# Autodesk Inventor assembly: 001_pakutta_all
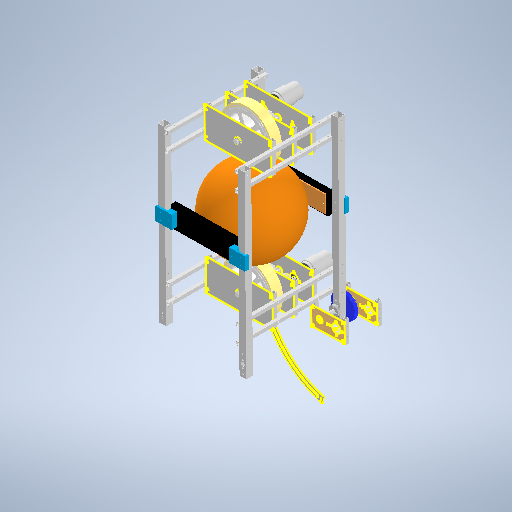
[picture p0: Inventor's stored thumbnail of the model, 512x512]
Saved by Autodesk Inventor 2025.1 (Build 291241000, 241)
## iProperties
Created: 2024-10-08
Part Number: 001_pakutta_all
Document SubType Name: Assembly
Designer: yuki0520
Author: yuki0520
## Documents named in this file (15)
- C:\Users\yuki0520\OneDrive\ドキュメント\Inventor\2025_nhk\tanaka\nageru\pakuriz\001_pakutta_all.iam
- C:\Users\yuki0520\OneDrive\ドキュメント\Inventor\2025_nhk\tanaka\nageru\pakuriz\001_pakutta_L.iam
- C:\Users\yuki0520\OneDrive\ドキュメント\Inventor\2025_nhk\tanaka\nageru\pakuriz\kaku_1010_530.ipt
- C:\Users\yuki0520\OneDrive\ドキュメント\Inventor\2025_nhk\tanaka\object\ball.ipt
- C:\Users\yuki0520\OneDrive\ドキュメント\Inventor\2025_nhk\tanaka\nageru\pakuriz\TH22_soroban_sn.ipt
- C:\Users\yuki0520\OneDrive\ドキュメント\Inventor\2025_nhk\tanaka\nageru\pakuriz\soroban_hold.ipt
- C:\Users\yuki0520\OneDrive\ドキュメント\Inventor\2025_nhk\tanaka\nageru\pakuriz\xx_giar_12x6.ipt
- C:\Users\yuki0520\OneDrive\ドキュメント\Inventor\2025_nhk\tanaka\nageru\pakuriz\xx_SSCSM12-8b.ipt
- C:\Users\yuki0520\OneDrive\ドキュメント\Inventor\2025_nhk\tanaka\nageru\pakuriz\xx_plate_motor.ipt
- C:\Users\yuki0520\OneDrive\ドキュメント\Inventor\2025_nhk\tanaka\nageru\pakuriz\xx_jiku_kakudo.ipt
- C:\Users\yuki0520\OneDrive\ドキュメント\Inventor\2025_nhk\tanaka\nageru\pakuriz\bear_12_18.ipt
- C:\Users\yuki0520\OneDrive\ドキュメント\Inventor\2025_nhk\tanaka\nageru\pakuriz\kaku_2020_465.ipt
- C:\Users\yuki0520\OneDrive\ドキュメント\Inventor\2025_nhk\tanaka\nageru\pakuriz\xxkaku_1010.ipt
- C:\Users\yuki0520\OneDrive\ドキュメント\Inventor\2025_nhk\tanaka\nageru\pakuriz\xx_memo.ipt
- C:\Users\yuki0520\OneDrive\ドキュメント\Inventor\2025_nhk\tanaka\nageru\pakuriz\xx_hojopipe.ipt
## Components (26 placed, 14 different names)
1. 001_pakutta_L:1 [sub-assembly] — 挿入:5, 挿入:6, 正接:1, 挿入:14, 挿入:38, 挿入:40, 挿入:41, 挿入:43
2. 001_pakutta_L:2 [sub-assembly] — 挿入:12, 挿入:13, 挿入:39, 挿入:42, 正接:4
3. kaku_1010_530:2 — 挿入:5, 挿入:6, 挿入:12, 挿入:15, 挿入:16
4. ball:1 — 正接:1, 正接:4, 正接:5
5. kaku_1010_530:3 — 挿入:13, 挿入:14, 挿入:21, 挿入:22, 挿入:36, 挿入:37
6. TH22_soroban_sn:1 — 挿入:23, 挿入:34
7. TH22_soroban_sn:2 — 挿入:19, 挿入:20, 正接:5
8. soroban_hold:1 — 挿入:20, 挿入:55
9. soroban_hold:2 — 挿入:15, 挿入:16, 挿入:19
10. soroban_hold:3 — 挿入:21, 挿入:22, 挿入:23
11. soroban_hold:4 — 挿入:34, 挿入:54
12. 平歯車1:1 — 挿入:35, メイト:3, 挿入:36, メイト:7
13. xx_SSCSM12-8b:1 — 挿入:35, メイト:3, メイト:10
14. xx_plate_motor:1 — メイト:5, メイト:6, 挿入:44, 挿入:45, 挿入:46, 挿入:47, フラッシュ:1, メイト:10
15. xx_jiku_kakudo:1 — メイト:4, メイト:5, メイト:7, メイト:8, メイト:9, フラッシュ:1
16. bear_12_18:1 — メイト:4, メイト:6
17. xx_SSCSM12-8b:2 — メイト:8, 挿入:37
18. xx_plate_motor:2 — メイト:9, 挿入:48, 挿入:49, 挿入:50, 挿入:51
19. kaku_2020_465:1 — 挿入:41, 挿入:42, 挿入:43, 挿入:55
20. kaku_2020_465:2 — 挿入:38, 挿入:39, 挿入:40, 挿入:54, 挿入:56, フラッシュ:2
21. xxkaku_1010:1 — 挿入:44, 挿入:45
22. xxkaku_1010:2 — 挿入:46, 挿入:47
23. xxkaku_1010:3 — 挿入:50, 挿入:51
24. xxkaku_1010:4 — 挿入:48, 挿入:49
25. xx_memo:1 — 正接:6, 正接:7, フラッシュ:2
26. xx_hojopipe:1 — 挿入:56, 正接:6, 正接:7
## Relationships (48: Insert 33, Mate 8, Tangent 5, Flush 2)
- 挿入:5 [Insert]: 001_pakutta_L:1 ↔ kaku_1010_530:2
- 挿入:6 [Insert]: 001_pakutta_L:1 ↔ kaku_1010_530:2
- 挿入:12 [Insert]: 001_pakutta_L:2 ↔ kaku_1010_530:2
- 正接:1 [Tangent]: 001_pakutta_L:1 ↔ ball:1
- 挿入:13 [Insert]: 001_pakutta_L:2 ↔ kaku_1010_530:3
- 挿入:14 [Insert]: 001_pakutta_L:1 ↔ kaku_1010_530:3
- 挿入:15 [Insert]: kaku_1010_530:2 ↔ soroban_hold:2
- 挿入:16 [Insert]: kaku_1010_530:2 ↔ soroban_hold:2
- 挿入:19 [Insert]: TH22_soroban_sn:2 ↔ soroban_hold:2
- 挿入:20 [Insert]: TH22_soroban_sn:2 ↔ soroban_hold:1
- 挿入:21 [Insert]: kaku_1010_530:3 ↔ soroban_hold:3
- 挿入:22 [Insert]: kaku_1010_530:3 ↔ soroban_hold:3
- 挿入:23 [Insert]: TH22_soroban_sn:1 ↔ soroban_hold:3
- 挿入:34 [Insert]: TH22_soroban_sn:1 ↔ soroban_hold:4
- 挿入:35 [Insert]: 平歯車1:1 ↔ xx_SSCSM12-8b:1
- メイト:3 [Mate]: 平歯車1:1 ↔ xx_SSCSM12-8b:1
- 挿入:36 [Insert]: kaku_1010_530:3 ↔ 平歯車1:1
- メイト:4 [Mate]: xx_jiku_kakudo:1 ↔ bear_12_18:1
- メイト:5 [Mate]: xx_plate_motor:1 ↔ xx_jiku_kakudo:1
- メイト:6 [Mate]: xx_plate_motor:1 ↔ bear_12_18:1
- メイト:7 [Mate]: 平歯車1:1 ↔ xx_jiku_kakudo:1
- メイト:8 [Mate]: xx_jiku_kakudo:1 ↔ xx_SSCSM12-8b:2
- 挿入:37 [Insert]: kaku_1010_530:3 ↔ xx_SSCSM12-8b:2
- メイト:9 [Mate]: xx_jiku_kakudo:1 ↔ xx_plate_motor:2
- 挿入:38 [Insert]: 001_pakutta_L:1 ↔ kaku_2020_465:2
- 挿入:39 [Insert]: 001_pakutta_L:2 ↔ kaku_2020_465:2
- 挿入:40 [Insert]: 001_pakutta_L:1 ↔ kaku_2020_465:2
- 挿入:41 [Insert]: 001_pakutta_L:1 ↔ kaku_2020_465:1
- 挿入:42 [Insert]: 001_pakutta_L:2 ↔ kaku_2020_465:1
- 挿入:43 [Insert]: 001_pakutta_L:1 ↔ kaku_2020_465:1
- 挿入:44 [Insert]: xx_plate_motor:1 ↔ xxkaku_1010:1
- 挿入:45 [Insert]: xx_plate_motor:1 ↔ xxkaku_1010:1
- 挿入:46 [Insert]: xx_plate_motor:1 ↔ xxkaku_1010:2
- 挿入:47 [Insert]: xx_plate_motor:1 ↔ xxkaku_1010:2
- 挿入:48 [Insert]: xx_plate_motor:2 ↔ xxkaku_1010:4
- 挿入:49 [Insert]: xx_plate_motor:2 ↔ xxkaku_1010:4
- 挿入:50 [Insert]: xx_plate_motor:2 ↔ xxkaku_1010:3
- 挿入:51 [Insert]: xx_plate_motor:2 ↔ xxkaku_1010:3
- 挿入:54 [Insert]: soroban_hold:4 ↔ kaku_2020_465:2
- 挿入:55 [Insert]: soroban_hold:1 ↔ kaku_2020_465:1
- 正接:4 [Tangent]: 001_pakutta_L:2 ↔ ball:1
- 正接:5 [Tangent]: ball:1 ↔ TH22_soroban_sn:2
- フラッシュ:1 [Flush] (-10 mm): xx_plate_motor:1 ↔ xx_jiku_kakudo:1
- メイト:10 [Mate] (10 mm): xx_SSCSM12-8b:1 ↔ xx_plate_motor:1
- 挿入:56 [Insert]: kaku_2020_465:2 ↔ xx_hojopipe:1
- 正接:6 [Tangent]: xx_memo:1 ↔ xx_hojopipe:1
- 正接:7 [Tangent]: xx_memo:1 ↔ xx_hojopipe:1
- フラッシュ:2 [Flush] (-5 mm): kaku_2020_465:2 ↔ xx_memo:1
